# Autodesk Inventor assembly: MainAssembly
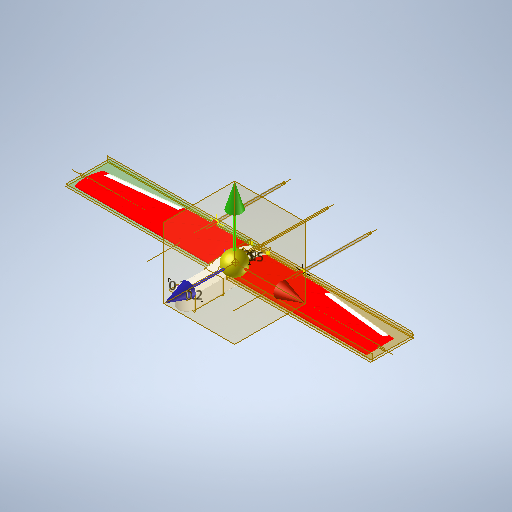
[picture p0: Inventor's stored thumbnail of the model, 512x512]
Saved by Autodesk Inventor 2026 (Build 300175050, 175E)
## iProperties
Created: 2025-08-01
Part Number: MainAssembly
Document SubType Name: Assembly
Designer: Cupri
Author: Cupri
## Documents named in this file (18)
- C:\Users\Cupri\OneDrive - University of South Carolina\Lab projects\UAV\SWIFT-UAV\System_development\Pelican\v0.2.1\MainAssembly\MainAssembly.iam
- C:\Users\Cupri\OneDrive - University of South Carolina\Lab projects\UAV\SWIFT-UAV\System_development\Pelican\v0.2.1\Parts\WingParts\WingBox.ipt
- C:\Users\Cupri\OneDrive - University of South Carolina\Lab projects\UAV\SWIFT-UAV\System_development\Pelican\v0.2.1\Parts\WingParts\WingLeft_v0.1.ipt
- C:\Users\Cupri\OneDrive - University of South Carolina\Lab projects\UAV\SWIFT-UAV\System_development\Pelican\v0.2.1\Parts\Extrusion\20x20x1295ExtrudedAluminum.ipt
- C:\Users\Cupri\OneDrive - University of South Carolina\Lab projects\UAV\SWIFT-UAV\System_development\Pelican\v0.2.1\Parts\Plates\2020 T Plate Bracket Connectors .ipt
- C:\Users\Cupri\OneDrive - University of South Carolina\Lab projects\UAV\SWIFT-UAV\System_development\Pelican\v0.2.1\Parts\Extrusion\20x20x800ExtrudedAluminum.ipt
- C:\Users\Cupri\OneDrive - University of South Carolina\Lab projects\UAV\SWIFT-UAV\System_development\Pelican\v0.2.1\Parts\Extrusion\20x20x130ExtrudedAluminum.ipt
- C:\Users\Cupri\OneDrive - University of South Carolina\Lab projects\UAV\SWIFT-UAV\System_development\Pelican\v0.2.1\Parts\AlerionLeft.ipt
- C:\Users\Cupri\OneDrive - University of South Carolina\Lab projects\UAV\SWIFT-UAV\System_development\Pelican\v0.2.1\Parts\WingParts\WingLeft_v0.1_MIR.ipt
- C:\Users\Cupri\OneDrive - University of South Carolina\Lab projects\UAV\SWIFT-UAV\System_development\Pelican\v0.2.1\Parts\Extrusion\20x20x1295ExtrudedAluminum_MIR1.ipt
- C:\Users\Cupri\OneDrive - University of South Carolina\Lab projects\UAV\SWIFT-UAV\System_development\Pelican\v0.2.1\Parts\Plates\2020 T Plate Bracket Connectors _MIR1.ipt
- C:\Users\Cupri\OneDrive - University of South Carolina\Lab projects\UAV\SWIFT-UAV\System_development\Pelican\v0.2.1\Parts\Extrusion\20x20x800ExtrudedAluminum_MIR1.ipt
- C:\Users\Cupri\OneDrive - University of South Carolina\Lab projects\UAV\SWIFT-UAV\System_development\Pelican\v0.2.1\Parts\AlerionLeft_MIR.ipt
- C:\Users\Cupri\OneDrive - University of South Carolina\Lab projects\UAV\SWIFT-UAV\System_development\Pelican\v0.2.1\Parts\WingBox.ipt
- C:\Users\Cupri\OneDrive - University of South Carolina\Lab projects\UAV\SWIFT-UAV\System_development\Pelican\v0.2.1\Parts\ForwardSection1.ipt
- C:\Users\Cupri\OneDrive - University of South Carolina\Lab projects\UAV\SWIFT-UAV\System_development\Pelican\v0.2.1\Parts\FrontSection2.ipt
- C:\Users\Cupri\OneDrive - University of South Carolina\Lab projects\UAV\SWIFT-UAV\System_development\Pelican\v0.2.1\Parts\Lid1.ipt
- C:\Users\Cupri\OneDrive - University of South Carolina\Lab projects\UAV\SWIFT-UAV\System_development\Pelican\v0.2.1\Parts\Lid2.ipt
## Components (19 placed, 16 different names)
1. WingBox:1 — Mate:1, Mate:4, Mate:12, Mate:13, Mate:29, Flush:5
2. WingLeft_v0.1:1 — Mate:1, Mate:2, Mate:3, Mate:4, Mate:5, Mate:8, Flush:1, Flush:2, Mate:17
3. 20x20x1295ExtrudedAluminum:1 — Mate:2, Mate:3, Mate:6, Mate:11, Mate:15
4. 2020 T Plate Bracket Connectors :1 — Mate:7, Mate:8, Mate:9, Mate:10
5. 2020 T Plate Bracket Connectors :2 — Mate:13, Mate:14, Mate:16
6. 20x20x800ExtrudedAluminum:1 — Mate:5, Mate:6, Mate:7, Mate:9, Mate:10, Mate:17
7. 20x20x130ExtrudedAluminum:1 — Mate:11, Mate:12, Mate:14, Mate:15, Mate:16, Mate:30, Mate:31, Flush:4
8. AlerionLeft:1 — Flush:1
9. WingLeft_v0.1_MIR:1 — Mate:18, Mate:19, Mate:20, Mate:21, Mate:26, Mate:27, Flush:3
10. 20x20x1295ExtrudedAluminum_MIR1:1 — Mate:18, Mate:19, Mate:25
11. 2020 T Plate Bracket Connectors _MIR1:1 — Mate:20, Mate:22, Mate:23, Mate:24
12. 20x20x800ExtrudedAluminum_MIR1:1 — Mate:21, Mate:22, Mate:23, Mate:24, Mate:25, Mate:26
13. AlerionLeft_MIR:1 — Mate:27
14. 2020 T Plate Bracket Connectors :3 — Mate:29, Mate:30, Mate:31, Flush:4
15. WingBox:2 — Flush:5, Flush:6
16. ForwardSection1:1 — Flush:6, Flush:7, Flush:8
17. FrontSection2:1 — Flush:7, Flush:9
18. Lid1:1 — Flush:8
19. Lid2:1 — Flush:9
## Relationships (39: Mate 30, Flush 9)
- Mate:1: WingBox:1 ↔ WingLeft_v0.1:1
- Mate:2: WingLeft_v0.1:1 ↔ 20x20x1295ExtrudedAluminum:1
- Mate:3: WingLeft_v0.1:1 ↔ 20x20x1295ExtrudedAluminum:1
- Mate:4: WingBox:1 ↔ WingLeft_v0.1:1
- Mate:5: WingLeft_v0.1:1 ↔ 20x20x800ExtrudedAluminum:1
- Mate:6: 20x20x1295ExtrudedAluminum:1 ↔ 20x20x800ExtrudedAluminum:1
- Mate:7: 2020 T Plate Bracket Connectors :1 ↔ 20x20x800ExtrudedAluminum:1
- Mate:8: WingLeft_v0.1:1 ↔ 2020 T Plate Bracket Connectors :1
- Mate:9: 2020 T Plate Bracket Connectors :1 ↔ 20x20x800ExtrudedAluminum:1
- Mate:10: 2020 T Plate Bracket Connectors :1 ↔ 20x20x800ExtrudedAluminum:1
- Mate:11: 20x20x1295ExtrudedAluminum:1 ↔ 20x20x130ExtrudedAluminum:1
- Mate:12: WingBox:1 ↔ 20x20x130ExtrudedAluminum:1
- Mate:13: WingBox:1 ↔ 2020 T Plate Bracket Connectors :2
- Mate:14: 2020 T Plate Bracket Connectors :2 ↔ 20x20x130ExtrudedAluminum:1
- Mate:15: 20x20x1295ExtrudedAluminum:1 ↔ 20x20x130ExtrudedAluminum:1
- Mate:16: 2020 T Plate Bracket Connectors :2 ↔ 20x20x130ExtrudedAluminum:1
- Flush:1: WingLeft_v0.1:1 ↔ AlerionLeft:1
- Flush:2: WingLeft_v0.1:1
- Mate:17: WingLeft_v0.1:1 ↔ 20x20x800ExtrudedAluminum:1
- Mate:18: WingLeft_v0.1_MIR:1 ↔ 20x20x1295ExtrudedAluminum_MIR1:1
- Mate:19: WingLeft_v0.1_MIR:1 ↔ 20x20x1295ExtrudedAluminum_MIR1:1
- Mate:20: WingLeft_v0.1_MIR:1 ↔ 2020 T Plate Bracket Connectors _MIR1:1
- Mate:21: WingLeft_v0.1_MIR:1 ↔ 20x20x800ExtrudedAluminum_MIR1:1
- Mate:22: 2020 T Plate Bracket Connectors _MIR1:1 ↔ 20x20x800ExtrudedAluminum_MIR1:1
- Mate:23: 2020 T Plate Bracket Connectors _MIR1:1 ↔ 20x20x800ExtrudedAluminum_MIR1:1
- Mate:24: 2020 T Plate Bracket Connectors _MIR1:1 ↔ 20x20x800ExtrudedAluminum_MIR1:1
- Mate:25: 20x20x1295ExtrudedAluminum_MIR1:1 ↔ 20x20x800ExtrudedAluminum_MIR1:1
- Mate:26: WingLeft_v0.1_MIR:1 ↔ 20x20x800ExtrudedAluminum_MIR1:1
- Mate:27: WingLeft_v0.1_MIR:1 ↔ AlerionLeft_MIR:1
- Flush:3: WingLeft_v0.1_MIR:1
- Mate:29: WingBox:1 ↔ 2020 T Plate Bracket Connectors :3
- Mate:30: 20x20x130ExtrudedAluminum:1 ↔ 2020 T Plate Bracket Connectors :3
- Mate:31: 20x20x130ExtrudedAluminum:1 ↔ 2020 T Plate Bracket Connectors :3
- Flush:4: 20x20x130ExtrudedAluminum:1 ↔ 2020 T Plate Bracket Connectors :3
- Flush:5: WingBox:1 ↔ WingBox:2
- Flush:6: WingBox:2 ↔ ForwardSection1:1
- Flush:7: ForwardSection1:1 ↔ FrontSection2:1
- Flush:8: ForwardSection1:1 ↔ Lid1:1
- Flush:9: FrontSection2:1 ↔ Lid2:1
